# Autodesk Inventor assembly: Assembly_TIRF_Smartphone_v0
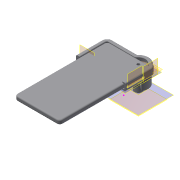
[picture p0: Inventor's stored thumbnail of the model, 180x180]
Saved by Autodesk Inventor 2019 (Build 230136000, 136)
## iProperties
Created: 2019-06-17
Part Number: Assembly_TIRF_Smartphone_v0
Document SubType Name: Assembly
Designer: diederichbenedict
Author: diederichbenedict
## Documents named in this file (6)
- C:\Users\diederichbenedict\Dropbox\Dokumente\Promotion\PROJECTS\STORMoChip\INVENTOR\Nanoscopy-on-a-cheap\Assembly_TIRF_Smartphone_v0.iam
- C:\Users\diederichbenedict\Dropbox\Dokumente\Promotion\PROJECTS\STORMoChip\INVENTOR\Nanoscopy-on-a-cheap\100_Huawei_P9.ipt
- C:\Users\diederichbenedict\Dropbox\Dokumente\Promotion\PROJECTS\STORMoChip\INVENTOR\Nanoscopy-on-a-cheap\100_CCTV_Fisheye_Starlight_f2.8mm_Fno_1.4.ipt
- C:\Users\diederichbenedict\Dropbox\Dokumente\Promotion\PROJECTS\STORMoChip\INVENTOR\Nanoscopy-on-a-cheap\100_chroma_HQ675_55.ipt
- C:\Users\diederichbenedict\Dropbox\Dokumente\Promotion\PROJECTS\STORMoChip\INVENTOR\Nanoscopy-on-a-cheap\100_Huawei_FilterLens_Adapter.ipt
- C:\Users\diederichbenedict\Dropbox\Dokumente\Promotion\PROJECTS\STORMoChip\INVENTOR\Nanoscopy-on-a-cheap\101_Huawei_FilterLens_Adapter_Thread.ipt
## Components (5 placed, 5 different names)
1. 100_Huawei_P9:1 — Insert:1, Mate:2, Mate:3, Angle:1
2. 100_CCTV_Fisheye_Starlight_f2.8mm_Fno_1.4:1 — Insert:2, Flush:3
3. 100_chroma_HQ675_55:1 — Insert:1, Insert:2
4. 100_Huawei_FilterLens_Adapter:1 — Mate:2, Mate:3, Angle:1, Flush:1, Flush:2
5. 101_Huawei_FilterLens_Adapter_Thread:1 — Flush:1, Flush:2, Flush:3
## Relationships (8: Flush 3, Insert 2, Mate 2, Angle 1)
- Insert:1 (0.3 mm): 100_Huawei_P9:1 ↔ 100_chroma_HQ675_55:1
- Insert:2 (2 mm): 100_CCTV_Fisheye_Starlight_f2.8mm_Fno_1.4:1 ↔ 100_chroma_HQ675_55:1
- Mate:2: 100_Huawei_P9:1 ↔ 100_Huawei_FilterLens_Adapter:1
- Mate:3: 100_Huawei_P9:1 ↔ 100_Huawei_FilterLens_Adapter:1
- Angle:1 (180 deg): 100_Huawei_P9:1 ↔ 100_Huawei_FilterLens_Adapter:1
- Flush:1: 100_Huawei_FilterLens_Adapter:1 ↔ 101_Huawei_FilterLens_Adapter_Thread:1
- Flush:2: 100_Huawei_FilterLens_Adapter:1 ↔ 101_Huawei_FilterLens_Adapter_Thread:1
- Flush:3: 100_CCTV_Fisheye_Starlight_f2.8mm_Fno_1.4:1 ↔ 101_Huawei_FilterLens_Adapter_Thread:1
